# Autodesk Inventor assembly: coffeeShop
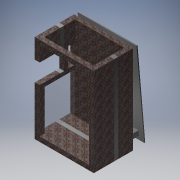
[picture p0: Inventor's stored thumbnail of the model, 180x180]
Saved by Autodesk Inventor 2019 (Build 230136000, 136)
## iProperties
Created: 2018-09-20
Part Number: coffeeShop
Document SubType Name: Assembly
Designer: wade
Author: wade
## Documents named in this file (3)
- C:\Users\wade\Documents\InventorParts\coffeeShop.iam
- C:\Users\wade\Documents\InventorParts\coffeeShopFrame.ipt
- C:\Users\wade\Documents\InventorParts\coffeeWindowFrontLeft.ipt
## Components (3 placed, 2 different names)
1. coffeeShopFrame:1 — Mate:1, Mate:2, Mate:3, Mate:7, Mate:8, Mate:9, Mate:10, Mate:11
2. coffeeWindowFrontLeft:1 — Mate:11, Mate:12, Mate:13
3. coffeeWindowFrontLeft:2 — Mate:4, Mate:5, Mate:6, Mate:7, Mate:8
## Relationships (14: Mate 14)
- Mate:1: coffeeShopFrame:1
- Mate:2: coffeeShopFrame:1
- Mate:3: coffeeShopFrame:1
- Mate:4: coffeeWindowFrontLeft:2
- Mate:5: coffeeWindowFrontLeft:2
- Mate:6: coffeeWindowFrontLeft:2
- Mate:7: coffeeShopFrame:1 ↔ coffeeWindowFrontLeft:2
- Mate:8: coffeeShopFrame:1 ↔ coffeeWindowFrontLeft:2
- Mate:9: coffeeShopFrame:1
- Mate:10: coffeeShopFrame:1
- Mate:11: coffeeShopFrame:1 ↔ coffeeWindowFrontLeft:1
- Mate:12: coffeeWindowFrontLeft:1
- Mate:13: coffeeWindowFrontLeft:1
- Mate:14
